# Autodesk Inventor assembly: exploration model
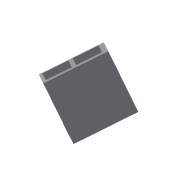
[picture p0: Inventor's stored thumbnail of the model, 180x180]
Saved by Autodesk Inventor 2019 (Build 230136000, 136)
## iProperties
Created: 2020-03-04
Part Number: exploration model
Document SubType Name: Assembly
Designer: Sandeep Shankar P
Author: Sandeep Shankar P
## Documents named in this file (3)
- C:\Users\Sandeep Shankar P\Documents\exploration model.iam
- C:\Users\Sandeep Shankar P\Documents\exploration1.ipt
- C:\Users\Sandeep Shankar P\Documents\exploration1.1.ipt
## Components (2 placed, 2 different names)
1. exploration1:1 — Rigid:1
2. exploration1.1:1 — Rigid:1
## Relationships (1: WeldJoint 1)
- Rigid:1 [WeldJoint]: exploration1:1 ↔ exploration1.1:1
